# Autodesk Inventor assembly: gear180_01
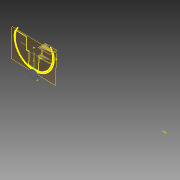
[picture p0: Inventor's stored thumbnail of the model, 180x180]
Saved by Autodesk Inventor 2013 (Build 170138000, 138)
## iProperties
Created: 2013-02-22
Part Number: gear180_01
Document SubType Name: Assembly
Designer: Nano
Author: Nano
## Documents named in this file (6)
- C:\Users\Nano\Documents\InventorByron\InventorMasterProject\gyroPhone01\gear180_01.iam
- C:\Users\Nano\Documents\InventorByron\InventorMasterProject\gyroPhone01\gear180mainBody01.ipt
- C:\Users\Nano\Documents\InventorByron\InventorMasterProject\gyroPhone01\gear180_01\Design Accelerator\Spur Gears1.iam
- C:\Users\Nano\Documents\InventorByron\InventorMasterProject\gyroPhone01\brace01.ipt
- C:\Users\Nano\Documents\InventorByron\InventorMasterProject\gyroPhone01\brace02.ipt
- C:\Users\Nano\Documents\InventorByron\InventorMasterProject\gyroPhone01\gearGuideRings.ipt
## Components (5 placed, 5 different names)
1. gear180mainBody01:1
2. Spur Gears:1 [sub-assembly] — Flush:1, Flush:2, Flush:3, Flush:4, Mate:1, Flush:6, Flush:7, Flush:8, Flush:9
3. brace01:1 — Flush:1, Flush:2, Flush:3, Flush:4
4. brace02:1 — Flush:5, Mate:1, Flush:6, Flush:7
5. gearGuideRings:1 — Flush:8, Flush:9
## Relationships (10: Flush 9, Mate 1)
- Flush:1: Spur Gears:1 ↔ brace01:1
- Flush:2: Spur Gears:1 ↔ brace01:1
- Flush:3: Spur Gears:1 ↔ brace01:1
- Flush:4: Spur Gears:1 ↔ brace01:1
- Flush:5: brace02:1
- Mate:1 (25.4 mm): Spur Gears:1 ↔ brace02:1
- Flush:6: Spur Gears:1 ↔ brace02:1
- Flush:7: Spur Gears:1 ↔ brace02:1
- Flush:8: Spur Gears:1 ↔ gearGuideRings:1
- Flush:9: Spur Gears:1 ↔ gearGuideRings:1
